# Autodesk Inventor assembly: ASSEMBLY_Y_Axis_Belt_Tensioner
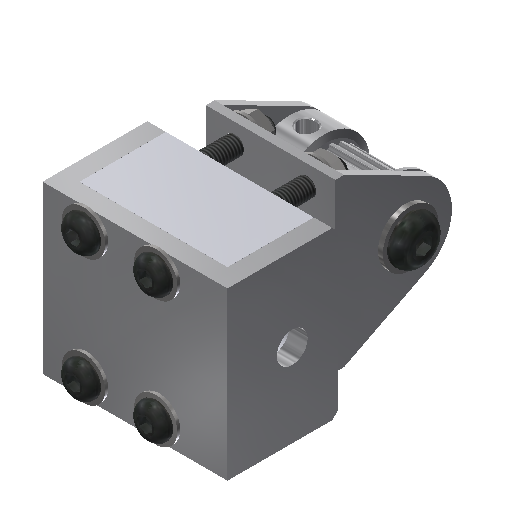
[picture p0: Inventor's stored thumbnail of the model, 512x512]
Saved by Autodesk Inventor 2026.1 (Build 301233000, 233)
## iProperties
Created: 2017-08-27
Part Number: ASSEMBLY_Y_Axis_Belt_Tensioner
Material: Ogólny
Document SubType Name: Assembly
Designer: Andrzej
Author: Andrzej
## Documents named in this file (12)
- C:\Users\Andrzej\OneDrive\_DRIVE_SYNCH_FILES\__ BYTECHLAB PROJECTS\MECH - FDM 3D Printer - RAPTOR-360\MCAD\1_REV1\ASSEMBLY_MAIN_REVA\ASSEMBLY_Y_Axis_Belt_Tensioner.iam
- C:\Users\Andrzej\OneDrive\_DRIVE_SYNCH_FILES\__ BYTECHLAB PROJECTS\MECH - FDM 3D Printer - RAPTOR-360\MCAD\1_REV1\__COTS_PARTS\COTS_GENERIC_GT2_20T_Pulley_8mm_Shaft.ipt
- C:\Users\Andrzej\OneDrive\_DRIVE_SYNCH_FILES\__ BYTECHLAB PROJECTS\MECH - FDM 3D Printer - RAPTOR-360\MCAD\1_REV1\__COTS_PARTS\COTS_GENERIC_SMR84ZZ_Bearing.ipt
- C:\Users\Andrzej\OneDrive\_DRIVE_SYNCH_FILES\__ BYTECHLAB PROJECTS\MECH - FDM 3D Printer - RAPTOR-360\MCAD\1_REV1\ASSEMBLY_MAIN_REVA\CNCM_Y_Axis_Tensioning_System_C_Sec_Idler.ipt
- C:\Users\Andrzej\OneDrive\_DRIVE_SYNCH_FILES\__ BYTECHLAB PROJECTS\MECH - FDM 3D Printer - RAPTOR-360\MCAD\1_REV1\ASSEMBLY_MAIN_REVA\CNCM_ALU_Y_Axis_Tensioning_System_C_Sec.ipt
- C:\Users\Andrzej\OneDrive\_DRIVE_SYNCH_FILES\__ BYTECHLAB PROJECTS\MECH - FDM 3D Printer - RAPTOR-360\MCAD\1_REV1\ASSEMBLY_MAIN_REVA\3DP_ABS_Y_Axis_Tenioning_System_C_Sec_Filler.ipt
- C:\Users\Andrzej\OneDrive\_DRIVE_SYNCH_FILES\__ BYTECHLAB PROJECTS\MECH - FDM 3D Printer - RAPTOR-360\MCAD\1_REV1\__CONTENT_CENTER_PARTS\en-US\DIN 125-1  A\DIN 125 - A 3,2.ipt
- C:\Users\Andrzej\OneDrive\_DRIVE_SYNCH_FILES\__ BYTECHLAB PROJECTS\MECH - FDM 3D Printer - RAPTOR-360\MCAD\1_REV1\__CONTENT_CENTER_PARTS\en-US\ISO 7380-1\ISO 7380-1 - M3 x 30.ipt
- C:\Users\Andrzej\OneDrive\_DRIVE_SYNCH_FILES\__ BYTECHLAB PROJECTS\MECH - FDM 3D Printer - RAPTOR-360\MCAD\1_REV1\__CONTENT_CENTER_PARTS\en-US\DIN 934\DIN 934 - M3 x 0,5.ipt
- C:\Users\Andrzej\OneDrive\_DRIVE_SYNCH_FILES\__ BYTECHLAB PROJECTS\MECH - FDM 3D Printer - RAPTOR-360\MCAD\1_REV1\__CONTENT_CENTER_PARTS\en-US\DIN 125-1  A\DIN 125 - A 4,3.ipt
- C:\Users\Andrzej\OneDrive\_DRIVE_SYNCH_FILES\__ BYTECHLAB PROJECTS\MECH - FDM 3D Printer - RAPTOR-360\MCAD\1_REV1\__CONTENT_CENTER_PARTS\en-US\ISO 7380-1\ISO 7380-1 - M4 x 25.ipt
- C:\Users\Andrzej\OneDrive\_DRIVE_SYNCH_FILES\__ BYTECHLAB PROJECTS\MECH - FDM 3D Printer - RAPTOR-360\MCAD\1_REV1\__CONTENT_CENTER_PARTS\en-US\DIN 934\DIN 934 - M4 x 0,7.ipt
## Components (29 placed, 11 different names)
1. COTS_GENERIC_GT2_20T_Pulley_8mm_Shaft:1 — Zestawiający:1, Zestawiający:3, Zestawiający:5, Zestawiający:7, Zestawiający:9, Równoległy:1, Zestawiający:11
2. COTS_GENERIC_SMR84ZZ_Bearing:1 — Zestawiający:1, Zestawiający:2, Zestawiający:10
3. COTS_GENERIC_SMR84ZZ_Bearing:2 — Zestawiający:2, Zestawiający:3, Zestawiający:4
4. COTS_GENERIC_SMR84ZZ_Bearing:3 — Zestawiający:4, Zestawiający:5, Zestawiający:6
5. COTS_GENERIC_SMR84ZZ_Bearing:4 — Zestawiający:6, Zestawiający:7, Zestawiający:8
6. COTS_GENERIC_SMR84ZZ_Bearing:5 — Zestawiający:8, Zestawiający:9, Równoległy:1
7. CNCM_Y_Axis_Tensioning_System_C_Sec_Idler:1 — Zestawiający:10, Zestawiający:11, Zestawiający:13, Równoległy:4, Zestawiający:14, Mate:24, Mate:26, Mate:28, Mate:30, Insert:9, Insert:10
8. CNCM_ALU_Y_Axis_Tensioning_System_C_Sec:1 — Zestawiający:12, Równoległy:2, Równoległy:3, Zestawiający:13, Równoległy:4, Zestawiający:14, Mate:15, Mate:16, Mate:17, Mate:18, Mate:19, Mate:20, Mate:21, Mate:22, Mate:23, Mate:25, Mate:27, Mate:29
9. 3DP_ABS_Y_Axis_Tenioning_System_C_Sec_Filler:1 — Zestawiający:12, Równoległy:2, Równoległy:3
10. DIN 125-1 A A 3,2:1 — Mate:15, Mate:16, Insert:1
11. ISO 7380-1 M3 x 30:1 — Insert:1
12. DIN 125-1 A A 3,2:2 — Mate:23, Mate:24, Insert:5
13. DIN 934 - replaced by DIN EN 24032/28673/28674 M3:1 — Insert:5
14. DIN 125-1 A A 3,2:3 — Mate:17, Mate:18, Insert:2
15. DIN 125-1 A A 3,2:4 — Mate:19, Mate:20, Insert:3
16. DIN 125-1 A A 3,2:5 — Mate:21, Mate:22, Insert:4
17. ISO 7380-1 M3 x 30:2 — Insert:2
18. ISO 7380-1 M3 x 30:3 — Insert:3
19. ISO 7380-1 M3 x 30:4 — Insert:4
20. DIN 125-1 A A 3,2:6 — Mate:25, Mate:26, Insert:6
21. DIN 125-1 A A 3,2:7 — Mate:27, Mate:28, Insert:7
22. DIN 125-1 A A 3,2:8 — Mate:29, Mate:30, Insert:8
23. DIN 934 - replaced by DIN EN 24032/28673/28674 M3:2 — Insert:6
24. DIN 934 - replaced by DIN EN 24032/28673/28674 M3:3 — Insert:7
25. DIN 934 - replaced by DIN EN 24032/28673/28674 M3:4 — Insert:8
26. DIN 125-1 A A 4,3:1 — Insert:9, Insert:12
27. DIN 125-1 A A 4,3:2 — Insert:10, Insert:11
28. ISO 7380-1 M4 x 25:1 — Insert:11
29. DIN 934 - replaced by DIN EN 24032/28673/28674 M4:1 — Insert:12
## Relationships (46: Mate 30, Insert 12, Flush 4)
- Zestawiający:1 [Mate]: COTS_GENERIC_GT2_20T_Pulley_8mm_Shaft:1 ↔ COTS_GENERIC_SMR84ZZ_Bearing:1
- Zestawiający:2 [Mate]: COTS_GENERIC_SMR84ZZ_Bearing:1 ↔ COTS_GENERIC_SMR84ZZ_Bearing:2
- Zestawiający:3 [Mate]: COTS_GENERIC_GT2_20T_Pulley_8mm_Shaft:1 ↔ COTS_GENERIC_SMR84ZZ_Bearing:2
- Zestawiający:4 [Mate]: COTS_GENERIC_SMR84ZZ_Bearing:2 ↔ COTS_GENERIC_SMR84ZZ_Bearing:3
- Zestawiający:5 [Mate]: COTS_GENERIC_GT2_20T_Pulley_8mm_Shaft:1 ↔ COTS_GENERIC_SMR84ZZ_Bearing:3
- Zestawiający:6 [Mate]: COTS_GENERIC_SMR84ZZ_Bearing:3 ↔ COTS_GENERIC_SMR84ZZ_Bearing:4
- Zestawiający:7 [Mate]: COTS_GENERIC_GT2_20T_Pulley_8mm_Shaft:1 ↔ COTS_GENERIC_SMR84ZZ_Bearing:4
- Zestawiający:8 [Mate]: COTS_GENERIC_SMR84ZZ_Bearing:4 ↔ COTS_GENERIC_SMR84ZZ_Bearing:5
- Zestawiający:9 [Mate]: COTS_GENERIC_GT2_20T_Pulley_8mm_Shaft:1 ↔ COTS_GENERIC_SMR84ZZ_Bearing:5
- Równoległy:1 [Flush] (1 mm): COTS_GENERIC_GT2_20T_Pulley_8mm_Shaft:1 ↔ COTS_GENERIC_SMR84ZZ_Bearing:5
- Zestawiający:10 [Mate]: COTS_GENERIC_SMR84ZZ_Bearing:1 ↔ CNCM_Y_Axis_Tensioning_System_C_Sec_Idler:1
- Zestawiający:11 [Mate] (0.6 mm): COTS_GENERIC_GT2_20T_Pulley_8mm_Shaft:1 ↔ CNCM_Y_Axis_Tensioning_System_C_Sec_Idler:1
- Zestawiający:12 [Mate]: CNCM_ALU_Y_Axis_Tensioning_System_C_Sec:1 ↔ 3DP_ABS_Y_Axis_Tenioning_System_C_Sec_Filler:1
- Równoległy:2 [Flush]: CNCM_ALU_Y_Axis_Tensioning_System_C_Sec:1 ↔ 3DP_ABS_Y_Axis_Tenioning_System_C_Sec_Filler:1
- Równoległy:3 [Flush]: CNCM_ALU_Y_Axis_Tensioning_System_C_Sec:1 ↔ 3DP_ABS_Y_Axis_Tenioning_System_C_Sec_Filler:1
- Zestawiający:13 [Mate] (6 mm): CNCM_Y_Axis_Tensioning_System_C_Sec_Idler:1 ↔ CNCM_ALU_Y_Axis_Tensioning_System_C_Sec:1
- Równoległy:4 [Flush]: CNCM_Y_Axis_Tensioning_System_C_Sec_Idler:1 ↔ CNCM_ALU_Y_Axis_Tensioning_System_C_Sec:1
- Zestawiający:14 [Mate]: CNCM_Y_Axis_Tensioning_System_C_Sec_Idler:1 ↔ CNCM_ALU_Y_Axis_Tensioning_System_C_Sec:1
- Mate:15: CNCM_ALU_Y_Axis_Tensioning_System_C_Sec:1 ↔ DIN 125-1 A A 3,2:1
- Mate:16: CNCM_ALU_Y_Axis_Tensioning_System_C_Sec:1 ↔ DIN 125-1 A A 3,2:1
- Mate:17: CNCM_ALU_Y_Axis_Tensioning_System_C_Sec:1 ↔ DIN 125-1 A A 3,2:3
- Mate:18: CNCM_ALU_Y_Axis_Tensioning_System_C_Sec:1 ↔ DIN 125-1 A A 3,2:3
- Mate:19: CNCM_ALU_Y_Axis_Tensioning_System_C_Sec:1 ↔ DIN 125-1 A A 3,2:4
- Mate:20: CNCM_ALU_Y_Axis_Tensioning_System_C_Sec:1 ↔ DIN 125-1 A A 3,2:4
- Mate:21: CNCM_ALU_Y_Axis_Tensioning_System_C_Sec:1 ↔ DIN 125-1 A A 3,2:5
- Mate:22: CNCM_ALU_Y_Axis_Tensioning_System_C_Sec:1 ↔ DIN 125-1 A A 3,2:5
- Insert:1: DIN 125-1 A A 3,2:1 ↔ ISO 7380-1 M3 x 30:1
- Insert:2: DIN 125-1 A A 3,2:3 ↔ ISO 7380-1 M3 x 30:2
- Insert:3: DIN 125-1 A A 3,2:4 ↔ ISO 7380-1 M3 x 30:3
- Insert:4: DIN 125-1 A A 3,2:5 ↔ ISO 7380-1 M3 x 30:4
- Mate:23: CNCM_ALU_Y_Axis_Tensioning_System_C_Sec:1 ↔ DIN 125-1 A A 3,2:2
- Mate:24: CNCM_Y_Axis_Tensioning_System_C_Sec_Idler:1 ↔ DIN 125-1 A A 3,2:2
- Mate:25: CNCM_ALU_Y_Axis_Tensioning_System_C_Sec:1 ↔ DIN 125-1 A A 3,2:6
- Mate:26: CNCM_Y_Axis_Tensioning_System_C_Sec_Idler:1 ↔ DIN 125-1 A A 3,2:6
- Mate:27: CNCM_ALU_Y_Axis_Tensioning_System_C_Sec:1 ↔ DIN 125-1 A A 3,2:7
- Mate:28: CNCM_Y_Axis_Tensioning_System_C_Sec_Idler:1 ↔ DIN 125-1 A A 3,2:7
- Mate:29: CNCM_ALU_Y_Axis_Tensioning_System_C_Sec:1 ↔ DIN 125-1 A A 3,2:8
- Mate:30: CNCM_Y_Axis_Tensioning_System_C_Sec_Idler:1 ↔ DIN 125-1 A A 3,2:8
- Insert:5: DIN 125-1 A A 3,2:2 ↔ DIN 934 - replaced by DIN EN 24032/28673/28674 M3:1
- Insert:6: DIN 125-1 A A 3,2:6 ↔ DIN 934 - replaced by DIN EN 24032/28673/28674 M3:2
- Insert:7: DIN 125-1 A A 3,2:7 ↔ DIN 934 - replaced by DIN EN 24032/28673/28674 M3:3
- Insert:8: DIN 125-1 A A 3,2:8 ↔ DIN 934 - replaced by DIN EN 24032/28673/28674 M3:4
- Insert:9: CNCM_Y_Axis_Tensioning_System_C_Sec_Idler:1 ↔ DIN 125-1 A A 4,3:1
- Insert:10: CNCM_Y_Axis_Tensioning_System_C_Sec_Idler:1 ↔ DIN 125-1 A A 4,3:2
- Insert:11: DIN 125-1 A A 4,3:2 ↔ ISO 7380-1 M4 x 25:1
- Insert:12: DIN 125-1 A A 4,3:1 ↔ DIN 934 - replaced by DIN EN 24032/28673/28674 M4:1
